# Autodesk Inventor assembly: каретка
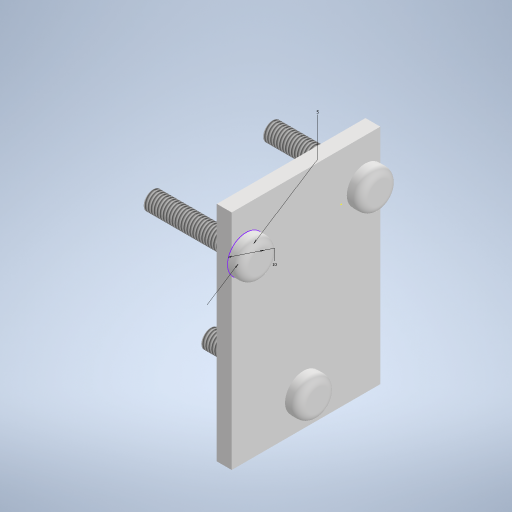
[picture p0: Inventor's stored thumbnail of the model, 512x512]
Saved by Autodesk Inventor 2024.2 (Build 282272000, 272)
## iProperties
Created: 2026-01-30
Part Number: каретка
Document SubType Name: Assembly
Designer: Service
Author: Service
## Documents named in this file (3)
- C:\Users\Service\Documents\Artist-v2\3D\каретка.iam
- C:\Users\Service\Documents\Основание.ipt
- C:\Users\Service\Documents\м5.ipt
## Components (4 placed, 2 different names)
1. Основание:1 — Заподлицо:1, Заподлицо:2, Совмещение:1, Совмещение:2, Совмещение:3, Совмещение:4, Совмещение:5
2. м5:1 — Заподлицо:1, Заподлицо:2, Совмещение:1
3. м5:2 — Совмещение:3, Совмещение:4
4. м5:3 — Совмещение:2, Совмещение:5
## Relationships (7: Mate 5, Flush 2)
- Заподлицо:1 [Flush]: Основание:1 ↔ м5:1
- Заподлицо:2 [Flush]: Основание:1 ↔ м5:1
- Совмещение:1 [Mate]: Основание:1 ↔ м5:1
- Совмещение:2 [Mate]: Основание:1 ↔ м5:3
- Совмещение:3 [Mate]: Основание:1 ↔ м5:2
- Совмещение:4 [Mate]: Основание:1 ↔ м5:2
- Совмещение:5 [Mate]: Основание:1 ↔ м5:3
